# Autodesk Inventor assembly: balboa-balancing-robot-kit
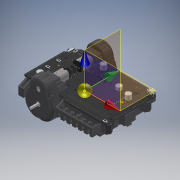
[picture p0: Inventor's stored thumbnail of the model, 180x180]
Saved by Autodesk Inventor 2018 (Build 220112000, 112)
## iProperties
Created: 2017-12-26
Part Number: balboa-balancing-robot-kit
Material: 一般
Description: STEP AP214
Document SubType Name: Assembly
Designer: ku_sk
Mass: 291.6 g
Surface Area: 949.804 cm^2
Volume: 138.841 cm^3
Density: 2.10025 g/cm^3
Sending System: SolidWorks 2016
Preprocessor: SwSTEP 2.0
Title: balboa-balancing-robot-kit.step
Revision Number: ANY
## Documents named in this file (3)
- D:\Inventor\Balboa32U4-CAD\Balboa32U4.iam
- D:\Inventor\Balboa32U4-CAD\parts\Body\Balboa32U4_Body.iam
- D:\Inventor\Balboa32U4-CAD\parts\Battery\Battery.iam
## Components (2 placed, 2 different names)
1. Balboa32U4_Body:1 [sub-assembly] — メイト:1, メイト:2, メイト:3, メイト:4, メイト:5, メイト:6
2. Battery:1 [sub-assembly] — メイト:4, メイト:5, メイト:6
## Relationships (6: Mate 6)
- メイト:1 [Mate]: Balboa32U4_Body:1
- メイト:2 [Mate]: Balboa32U4_Body:1
- メイト:3 [Mate]: Balboa32U4_Body:1
- メイト:4 [Mate]: Balboa32U4_Body:1 ↔ Battery:1
- メイト:5 [Mate]: Balboa32U4_Body:1 ↔ Battery:1
- メイト:6 [Mate]: Balboa32U4_Body:1 ↔ Battery:1
